# Autodesk Inventor assembly: cover2
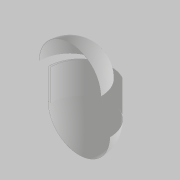
[picture p0: Inventor's stored thumbnail of the model, 180x180]
Saved by Autodesk Inventor 2021 (Build 250183000, 183)
## iProperties
Created: 2021-05-31
Part Number: cover2
Document SubType Name: Assembly
Designer: Watchdog
Author: Watchdog
## Documents named in this file (4)
- C:\Users\Watchdog\OneDrive - Flinders\Advn Mech Design Shared\6_Development\2_Design\inventor\cover\cover2.iam
- C:\Users\Watchdog\OneDrive - Flinders\Advn Mech Design Shared\6_Development\2_Design\inventor\cover\cover2_end.ipt
- C:\Users\Watchdog\OneDrive - Flinders\Advn Mech Design Shared\6_Development\2_Design\inventor\cover\cover2_shell_large.ipt
- C:\Users\Watchdog\OneDrive - Flinders\Advn Mech Design Shared\6_Development\2_Design\inventor\cover\cover2_shell_small.ipt
## Components (4 placed, 3 different names)
1. cover2_end:1 — Mate:1, Mate:2, Flush:1, Flush:2
2. cover2_shell_large:1 — Mate:1, Flush:1, Flush:3, Flush:4, Mate:3, Flush:5
3. cover2_shell_small:1 — Flush:3, Flush:4
4. cover2_end:2 — Mate:3, Flush:5
## Relationships (8: Flush 5, Mate 3)
- Mate:1: cover2_end:1 ↔ cover2_shell_large:1
- Mate:2: cover2_end:1
- Flush:1: cover2_end:1 ↔ cover2_shell_large:1
- Flush:2: cover2_end:1
- Flush:3: cover2_shell_large:1 ↔ cover2_shell_small:1
- Flush:4: cover2_shell_large:1 ↔ cover2_shell_small:1
- Mate:3: cover2_shell_large:1 ↔ cover2_end:2
- Flush:5: cover2_shell_large:1 ↔ cover2_end:2
